# Autodesk Inventor assembly: Ocean-Kostra-B
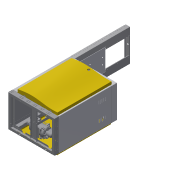
[picture p0: Inventor's stored thumbnail of the model, 180x180]
Saved by Autodesk Inventor 2017 (Build 210142000, 142)
## iProperties
Created: 2014-02-17
Part Number: Ocean-Kostra-B
Document SubType Name: Assembly
Designer: Евтушенко
Author: Евтушенко
## Documents named in this file (14)
- D:\ИНИТ\Разработка\Терминалы\Express Pos Cash v.2\00 - Прочее\OCEAN-36-WAVE\Ocean-Kostra-B.iam
- D:\ИНИТ\Разработка\Терминалы\Express Pos Cash v.2\00 - Прочее\OCEAN-36-WAVE\1756-211.iam
- D:\ИНИТ\Разработка\Терминалы\Express Pos Cash v.2\00 - Прочее\OCEAN-36-WAVE\K102-220-1562.iam
- D:\ИНИТ\Разработка\Терминалы\Express Pos Cash v.2\00 - Прочее\OCEAN-36-WAVE\K101-220-1562.iam
- D:\ИНИТ\Разработка\Терминалы\Express Pos Cash v.2\00 - Прочее\OCEAN-36-WAVE\1808-211.iam
- D:\ИНИТ\Разработка\Терминалы\Express Pos Cash v.2\00 - Прочее\OCEAN-36-WAVE\1770-211.iam
- D:\ИНИТ\Разработка\Терминалы\Express Pos Cash v.2\00 - Прочее\OCEAN-36-WAVE\2511-311.ipt
- D:\ИНИТ\Разработка\Терминалы\Express Pos Cash v.2\00 - Прочее\OCEAN-36-WAVE\1514-211_LITE.iam
- D:\ИНИТ\Разработка\Терминалы\Express Pos Cash v.2\00 - Прочее\OCEAN-36-WAVE\2639-411.ipt
- D:\ИНИТ\Разработка\Терминалы\Express Pos Cash v.2\00 - Прочее\OCEAN-36-WAVE\1675-311.iam
- D:\ИНИТ\Разработка\Терминалы\Express Pos Cash v.2\00 - Прочее\OCEAN-36-WAVE\1533-211.iam
- D:\ИНИТ\Разработка\Терминалы\Express Pos Cash v.2\00 - Прочее\OCEAN-36-WAVE\2561-312.iam
- D:\ИНИТ\Разработка\Терминалы\Express Pos Cash v.2\00 - Прочее\OCEAN-36-WAVE\M002330.ipt
- D:\ИНИТ\Разработка\Терминалы\Express Pos Cash v.2\00 - Прочее\OCEAN-36-WAVE\2570-311_TOP-DESIGN.ipt
## Components (14 placed, 13 different names)
1. 1756-211:1 [sub-assembly] — Совмещение:1
2. K102-220-1562:1 [sub-assembly]
3. K101-220-1562:1 [sub-assembly]
4. 1808-211:1 [sub-assembly] — Совмещение:2
5. 1770-211:1 [sub-assembly]
6. 2511-311:1
7. 1514-211_LITE:1 [sub-assembly] — Заподлицо:1, Совмещение:1, Совмещение:2, Заподлицо:2, Заподлицо:3
8. 2639-411:1
9. 1675-311:1 [sub-assembly]
10. 1675-311:4 [sub-assembly]
11. 1533-211:1 [sub-assembly] — Заподлицо:1, Заподлицо:2, Заподлицо:3
12. 2561-312:1 [sub-assembly]
13. M002330:1
14. 2570-311_TOP-DESIGN:1
## Relationships (5: Flush 3, Mate 2)
- Заподлицо:1 [Flush]: 1514-211_LITE:1 ↔ 1533-211:1
- Совмещение:1 [Mate] (-1010 mm): 1756-211:1 ↔ 1514-211_LITE:1
- Совмещение:2 [Mate]: 1808-211:1 ↔ 1514-211_LITE:1
- Заподлицо:2 [Flush]: 1514-211_LITE:1 ↔ 1533-211:1
- Заподлицо:3 [Flush]: 1514-211_LITE:1 ↔ 1533-211:1
